# Autodesk Inventor assembly: WingAssembly
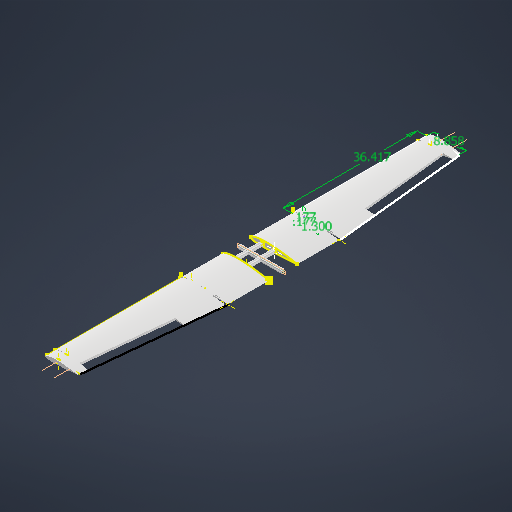
[picture p0: Inventor's stored thumbnail of the model, 512x512]
Saved by Autodesk Inventor 2026 (Build 300175050, 175E)
## iProperties
Created: 2025-06-04
Part Number: WingAssembly
Document SubType Name: Assembly
Designer: Cupri
Author: Cupri
## Documents named in this file (10)
- C:\Users\Cupri\OneDrive - University of South Carolina\Lab projects\UAV\SWIFT-UAV\System_development\Pelican\v0.2\SubAssemblies\WingAssembly\WingAssembly.iam
- C:\Users\Cupri\OneDrive - University of South Carolina\Lab projects\UAV\SWIFT-UAV\System_development\Pelican\v0.2\Parts\OuterWingRight.ipt
- C:\Users\Cupri\OneDrive - University of South Carolina\Lab projects\UAV\SWIFT-UAV\System_development\Pelican\v0.2\Parts\OuterWingRightCap.ipt
- C:\Users\Cupri\OneDrive - University of South Carolina\Lab projects\UAV\SWIFT-UAV\System_development\Pelican\v0.2\Parts\Extrusion\20x20x1300ExtrudedAluminum.ipt
- C:\Users\Cupri\OneDrive - University of South Carolina\Lab projects\UAV\SWIFT-UAV\System_development\Pelican\v0.2\Parts\Extrusion\20x20x300ExtrudedAluminum.ipt
- C:\Users\Cupri\OneDrive - University of South Carolina\Lab projects\UAV\SWIFT-UAV\System_development\Pelican\v0.2\Parts\MiddleWingRight.ipt
- C:\Users\Cupri\OneDrive - University of South Carolina\Lab projects\UAV\SWIFT-UAV\System_development\Pelican\v0.2\Parts\Extrusion\20x20x375ExtrudedAluminum.ipt
- C:\Users\Cupri\OneDrive - University of South Carolina\Lab projects\UAV\SWIFT-UAV\System_development\Pelican\v0.2\Parts\OuterWingLeft.ipt
- C:\Users\Cupri\OneDrive - University of South Carolina\Lab projects\UAV\SWIFT-UAV\System_development\Pelican\v0.2\Parts\OuterWingRightCapLeft.ipt
- C:\Users\Cupri\OneDrive - University of South Carolina\Lab projects\UAV\SWIFT-UAV\System_development\Pelican\v0.2\Parts\MiddleWingLeft.ipt
## Components (11 placed, 9 different names)
1. OuterWingRight:1 — Mate:10, Mate:11, Mate:15
2. OuterWingRightCap:1 — Mate:8, Mate:9, Mate:10, Mate:11
3. 20x20x1300ExtrudedAluminum:1 — Mate:6, Mate:8, Mate:9, Mate:14, Flush:4, Flush:6
4. 20x20x300ExtrudedAluminum:1 — Mate:6, Mate:17, Flush:3, Flush:4, Flush:6, Mate:18, Angle:1
5. MiddleWingRight:2 — Mate:14, Mate:15, Mate:16
6. 20x20x375ExtrudedAluminum:1 — Mate:16, Mate:17, Flush:3
7. OuterWingLeft:1 — Mate:20, Mate:21, Mate:24
8. OuterWingRightCapLeft:1 — Mate:20, Mate:21, Mate:22, Mate:23
9. 20x20x1300ExtrudedAluminum:2 — Mate:22, Mate:23, Mate:25
10. MiddleWingLeft:1 — Mate:24, Mate:25
11. 20x20x375ExtrudedAluminum:2
## Relationships (21: Mate 17, Flush 3, Angle 1)
- Mate:6: 20x20x1300ExtrudedAluminum:1 ↔ 20x20x300ExtrudedAluminum:1
- Mate:8: OuterWingRightCap:1 ↔ 20x20x1300ExtrudedAluminum:1
- Mate:9: OuterWingRightCap:1 ↔ 20x20x1300ExtrudedAluminum:1
- Mate:10: OuterWingRight:1 ↔ OuterWingRightCap:1
- Mate:11: OuterWingRight:1 ↔ OuterWingRightCap:1
- Mate:14: 20x20x1300ExtrudedAluminum:1 ↔ MiddleWingRight:2
- Mate:15: OuterWingRight:1 ↔ MiddleWingRight:2
- Mate:16: MiddleWingRight:2 ↔ 20x20x375ExtrudedAluminum:1
- Mate:17: 20x20x300ExtrudedAluminum:1 ↔ 20x20x375ExtrudedAluminum:1
- Flush:3: 20x20x300ExtrudedAluminum:1 ↔ 20x20x375ExtrudedAluminum:1
- Flush:4: 20x20x1300ExtrudedAluminum:1 ↔ 20x20x300ExtrudedAluminum:1
- Flush:6 (50.8 mm): 20x20x1300ExtrudedAluminum:1 ↔ 20x20x300ExtrudedAluminum:1
- Mate:18: 20x20x300ExtrudedAluminum:1
- Mate:19
- Angle:1 (-360 deg): 20x20x300ExtrudedAluminum:1
- Mate:20: OuterWingLeft:1 ↔ OuterWingRightCapLeft:1
- Mate:21: OuterWingLeft:1 ↔ OuterWingRightCapLeft:1
- Mate:22: OuterWingRightCapLeft:1 ↔ 20x20x1300ExtrudedAluminum:2
- Mate:23: OuterWingRightCapLeft:1 ↔ 20x20x1300ExtrudedAluminum:2
- Mate:24: OuterWingLeft:1 ↔ MiddleWingLeft:1
- Mate:25: 20x20x1300ExtrudedAluminum:2 ↔ MiddleWingLeft:1
